# Autodesk Inventor assembly: Oktagon Zusammenbau
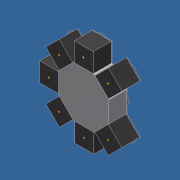
[picture p0: Inventor's stored thumbnail of the model, 180x180]
Saved by Autodesk Inventor 2018.2 (Build 222227000, 227)
## iProperties
Company: Fraunhofer ILT
Created: 2018-10-15
Part Number: Oktagon Zusammenbau
Material: geeigneten Werkstoff auswählen !
Document SubType Name: Assembly
Designer: N.Grubert
Title: =Description
Author: N.Grubert
## Documents named in this file (3)
- C:\Users\GRUBERT\Documents\COSIMA-Laserstar\CAD\Oktagon Zusammenbau.iam
- C:\Users\GRUBERT\Documents\COSIMA-Laserstar\CAD\Arduino_Oktagon.iam
- C:\Users\GRUBERT\Documents\COSIMA-Laserstar\CAD\Modul.iam
## Components (8 placed, 2 different names)
1. Arduino_Oktagon:1 [sub-assembly] — Passend:1, Passend:2, Passend:3, Passend:4, Passend:5, Passend:6, Passend:7, Passend:8, Passend:9, Passend:10, Fluchtend:1, Fluchtend:2, Fluchtend:3, Fluchtend:4, Fluchtend:5, Fluchtend:6, Fluchtend:7, Fluchtend:8
2. Modul:1 [sub-assembly] — Passend:4, Fluchtend:6
3. Modul:2 [sub-assembly] — Passend:5, Fluchtend:7
4. Modul:3 [sub-assembly] — Passend:6, Fluchtend:1, Fluchtend:8
5. Modul:4 [sub-assembly] — Passend:7, Fluchtend:2
6. Modul:5 [sub-assembly] — Passend:8, Fluchtend:3
7. Modul:6 [sub-assembly] — Passend:9, Fluchtend:4
8. Modul:7 [sub-assembly] — Passend:10, Fluchtend:5
## Relationships (18: Mate 10, Flush 8)
- Passend:1 [Mate]: Arduino_Oktagon:1
- Passend:2 [Mate]: Arduino_Oktagon:1
- Passend:3 [Mate]: Arduino_Oktagon:1
- Passend:4 [Mate]: Arduino_Oktagon:1 ↔ Modul:1
- Passend:5 [Mate]: Arduino_Oktagon:1 ↔ Modul:2
- Passend:6 [Mate]: Arduino_Oktagon:1 ↔ Modul:3
- Passend:7 [Mate]: Arduino_Oktagon:1 ↔ Modul:4
- Passend:8 [Mate]: Arduino_Oktagon:1 ↔ Modul:5
- Passend:9 [Mate]: Arduino_Oktagon:1 ↔ Modul:6
- Passend:10 [Mate]: Arduino_Oktagon:1 ↔ Modul:7
- Fluchtend:1 [Flush]: Arduino_Oktagon:1 ↔ Modul:3
- Fluchtend:2 [Flush]: Arduino_Oktagon:1 ↔ Modul:4
- Fluchtend:3 [Flush]: Arduino_Oktagon:1 ↔ Modul:5
- Fluchtend:4 [Flush]: Arduino_Oktagon:1 ↔ Modul:6
- Fluchtend:5 [Flush]: Arduino_Oktagon:1 ↔ Modul:7
- Fluchtend:6 [Flush]: Arduino_Oktagon:1 ↔ Modul:1
- Fluchtend:7 [Flush]: Arduino_Oktagon:1 ↔ Modul:2
- Fluchtend:8 [Flush]: Arduino_Oktagon:1 ↔ Modul:3
